# Autodesk Inventor assembly: F and B arm assembly
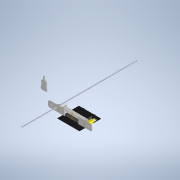
[picture p0: Inventor's stored thumbnail of the model, 180x180]
Saved by Autodesk Inventor 2021 (Build 250183000, 183)
## iProperties
Created: 2022-05-21
Part Number: F and B arm assembly
Document SubType Name: Assembly
Designer: techv
Author: techv
## Documents named in this file (12)
- D:\Projects\P_Baker Bot\Design\F and B assembly\F and B arm assembly.iam
- D:\Projects\P_Baker Bot\Design\F and B assembly\poly carbonate plate.ipt
- D:\Projects\P_Baker Bot\Design\F and B assembly\arm1.ipt
- D:\Projects\P_Baker Bot\Design\F and B assembly\Roller.ipt
- D:\Projects\P_Baker Bot\Design\F and B assembly\arm2.ipt
- D:\Projects\A_Electronics CAD model\BO DC Motor.ipt
- D:\Projects\P_Baker Bot\Design\F and B assembly\3d mount for linear bearing.ipt
- D:\Projects\P_Baker Bot\Design\F and B assembly\3d mount for linear bearing and leadscrew.ipt
- D:\Projects\P_Baker Bot\Design\F and B assembly\Linear_rod_nut_8mm.ipt
- D:\Projects\P_Baker Bot\Design\F and B assembly\spatula.ipt
- C:\Users\techv\Downloads\1M_8mm_2mm_4_start_Acme.ipt
- C:\Users\techv\Documents\learn bearing mount.ipt
## Components (12 placed, 11 different names)
1. poly carbonate plate:1 — Mate:34
2. Roller:1 — Mate:29, Mate:30, Mate:31, Mate:33
3. arm1:1 — Flush:5, Flush:6, Flush:7, Flush:8, Mate:14, Flush:12, Mate:16, Mate:20, Mate:21, Mate:25, Mate:28
4. arm2:1 — Flush:5, Flush:6, Mate:14, Mate:17
5. arm2:2 — Flush:7, Flush:8, Mate:24, Flush:14, Mate:28, Mate:29, Mate:32, Angle:2, Mate:34
6. BO DC Motor:1 — Mate:30, Mate:31, Mate:32, Mate:33, Angle:2
7. 3d mount for linear bearing:1 — Angle:1, Mate:24, Mate:25, Flush:14
8. 3d mount for linear bearing and leadscrew:1 — Flush:12, Mate:16, Mate:17, Mate:18, Mate:19
9. Linear_rod_nut_8mm:1 — Mate:18, Mate:19, Rotation:1, Mate:23
10. spatula:1 — Mate:20, Angle:1, Mate:21
11. 1M_8mm_2mm_4_start_Acme:1 — Rotation:1, Mate:23
12. learn bearing mount:1
## Relationships (26: Mate 17, Flush 6, Angle 2, RelateRotation 1)
- Flush:5: arm1:1 ↔ arm2:1
- Flush:6: arm1:1 ↔ arm2:1
- Flush:7: arm1:1 ↔ arm2:2
- Flush:8: arm1:1 ↔ arm2:2
- Mate:14: arm1:1 ↔ arm2:1
- Flush:12: arm1:1 ↔ 3d mount for linear bearing and leadscrew:1
- Mate:16: arm1:1 ↔ 3d mount for linear bearing and leadscrew:1
- Mate:17: arm2:1 ↔ 3d mount for linear bearing and leadscrew:1
- Mate:18: 3d mount for linear bearing and leadscrew:1 ↔ Linear_rod_nut_8mm:1
- Mate:19: 3d mount for linear bearing and leadscrew:1 ↔ Linear_rod_nut_8mm:1
- Mate:20: arm1:1 ↔ spatula:1
- Angle:1 (0 deg): 3d mount for linear bearing:1 ↔ spatula:1
- Mate:21: arm1:1 ↔ spatula:1
- Rotation:1 [RelateRotation] (0.988 ul): Linear_rod_nut_8mm:1 ↔ 1M_8mm_2mm_4_start_Acme:1
- Mate:23: Linear_rod_nut_8mm:1 ↔ 1M_8mm_2mm_4_start_Acme:1
- Mate:24: arm2:2 ↔ 3d mount for linear bearing:1
- Mate:25: arm1:1 ↔ 3d mount for linear bearing:1
- Flush:14: arm2:2 ↔ 3d mount for linear bearing:1
- Mate:28: arm1:1 ↔ arm2:2
- Mate:29: Roller:1 ↔ arm2:2
- Mate:30: Roller:1 ↔ BO DC Motor:1
- Mate:31: Roller:1 ↔ BO DC Motor:1
- Mate:32 (1.9 mm): arm2:2 ↔ BO DC Motor:1
- Mate:33: Roller:1 ↔ BO DC Motor:1
- Angle:2 (0 deg): arm2:2 ↔ BO DC Motor:1
- Mate:34 (7 mm): poly carbonate plate:1 ↔ arm2:2
